# Autodesk Inventor assembly: Gripper_for_Illustrations_fingers_only
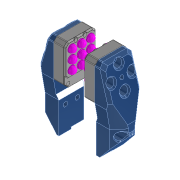
[picture p0: Inventor's stored thumbnail of the model, 180x180]
Saved by Autodesk Inventor 2022 (Build 260153000, 153)
## iProperties
Created: 2021-07-25
Part Number: Gripper_for_Illustrations_fingers_only
Document SubType Name: Assembly
Designer: exllu
Author: exllu
## Documents named in this file (10)
- C:\Users\kylem\OneDrive\Documents\GitHub\IMML_Contactile_Gripper_Hardware\Gripper_for_Illustrations_fingers_only.iam
- C:\Users\kylem\OneDrive\Documents\GitHub\IMML_Contactile_Gripper_Hardware\Compliant_plate.ipt
- C:\Users\kylem\OneDrive\Documents\GitHub\IMML_Contactile_Gripper_Hardware\Padding.ipt
- C:\Users\kylem\OneDrive\Documents\GitHub\IMML_Contactile_Gripper_Hardware\UR5_Mounting_Plate.ipt
- C:\Users\kylem\OneDrive\Documents\GitHub\IMML_Contactile_Gripper_Hardware\Contactile Communication Hub.ipt
- C:\Users\kylem\OneDrive\Documents\GitHub\IMML_Contactile_Gripper_Hardware\Finger Assembly Left.iam
- C:\Users\kylem\OneDrive\Documents\GitHub\IMML_Contactile_Gripper_Hardware\Finger Assembly Right.iam
- C:\Users\kylem\OneDrive\Documents\GitHub\IMML_Contactile_Gripper_Hardware\Contactile_Sensor.ipt
- C:\Users\kylem\OneDrive\Documents\GitHub\IMML_Contactile_Gripper_Hardware\camera_mount_v3.ipt
- C:\Users\kylem\OneDrive\Documents\GitHub\IMML_Contactile_Gripper_Hardware\camera_v2.ipt
## Components (10 placed, 9 different names)
1. Compliant_plate:1 — Mate:139
2. Padding:1 — Mate:139
3. UR5_Mounting_Plate:1
4. Contactile Communication Hub:1
5. Finger Assembly Right:1 [sub-assembly] — Mate:279
6. Finger Assembly Left:1 [sub-assembly] — Mate:275
7. Contactile_Sensor:1 — Mate:279
8. Contactile_Sensor:2 — Mate:275
9. camera_mount_v3:1 — Angle:4, Flush:61
10. camera_v2:1 — Angle:4, Flush:61
## Relationships (5: Mate 3, Angle 1, Flush 1)
- Mate:139: Compliant_plate:1 ↔ Padding:1
- Mate:275: Finger Assembly Left:1 ↔ Contactile_Sensor:2
- Mate:279: Finger Assembly Right:1 ↔ Contactile_Sensor:1
- Angle:4 (0 deg): camera_mount_v3:1 ↔ camera_v2:1
- Flush:61: camera_mount_v3:1 ↔ camera_v2:1
